# Autodesk Inventor assembly: Wheel Assembly
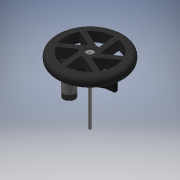
[picture p0: Inventor's stored thumbnail of the model, 180x180]
Saved by Autodesk Inventor 2017 (Build 210142000, 142)
## iProperties
Created: 2018-10-18
Part Number: Wheel Assembly
Document SubType Name: Assembly
Designer: Dell
Author: Dell
## Documents named in this file (8)
- C:\Users\Dell\Documents\GitHub\tr2\Wheel Assembly\Wheel Assembly.iam
- C:\Users\Dell\Documents\GitHub\tr2\Wheel Assembly\8mm Shaft.ipt
- C:\Users\Dell\Documents\GitHub\tr2\Wheel Assembly\Scooter Wheel.ipt
- C:\Users\Dell\Documents\GitHub\tr2\Wheel Assembly\WA01.ipt
- C:\Users\Dell\Documents\GitHub\tr2\Wheel Assembly\Wheel Assembly\Design Accelerator\Spur Gears1.iam
- C:\Users\Dell\Documents\GitHub\tr2\Base\37d-gearmotor-50-70-encoder.ipt
- C:\Users\Dell\Documents\GitHub\tr2\Wheel Assembly\22x8x8mm Bearing.ipt
- C:\Users\Dell\Documents\GitHub\tr2\Wheel Assembly\6mm Mounting Hub, thin.ipt
## Components (11 placed, 7 different names)
1. Scooter Wheel:1 — Mate:8, Flush:1, Mate:25, Mate:26, Mate:27, Mate:28
2. WA01:1 — Mate:2, Mate:9, Mate:10, Mate:11, Mate:24, Mate:31, Mate:33
3. 8mm Shaft:2 — Mate:2, Flush:1, Mate:16, Mate:18, Mate:23, Mate:29, Mate:30
4. Spur Gears:1 [sub-assembly] — Mate:8, Mate:17, Mate:19, Mate:21, Mate:22, Mate:30, Mate:31, Mate:32, Mate:33
5. 37d-gearmotor-50-70-encoder:1 — Mate:9, Mate:10, Mate:11, Mate:20, Mate:32
6. 22x8x8mm Bearing:1 — Mate:16, Mate:17
7. 22x8x8mm Bearing:2 — Mate:18, Mate:19
8. 6mm Mounting Hub, thin:1 — Mate:20, Mate:21, Mate:22
9. 22x8x8mm Bearing:3 — Mate:23, Mate:24
10. 22x8x8mm Bearing:4 — Mate:25, Mate:26
11. 22x8x8mm Bearing:5 — Mate:27, Mate:28, Mate:29
## Relationships (24: Mate 23, Flush 1)
- Mate:2: WA01:1 ↔ 8mm Shaft:2
- Mate:8: Scooter Wheel:1 ↔ Spur Gears:1
- Flush:1: Scooter Wheel:1 ↔ 8mm Shaft:2
- Mate:9: WA01:1 ↔ 37d-gearmotor-50-70-encoder:1
- Mate:10: WA01:1 ↔ 37d-gearmotor-50-70-encoder:1
- Mate:11: WA01:1 ↔ 37d-gearmotor-50-70-encoder:1
- Mate:16: 8mm Shaft:2 ↔ 22x8x8mm Bearing:1
- Mate:17: Spur Gears:1 ↔ 22x8x8mm Bearing:1
- Mate:18: 8mm Shaft:2 ↔ 22x8x8mm Bearing:2
- Mate:19: Spur Gears:1 ↔ 22x8x8mm Bearing:2
- Mate:20: 37d-gearmotor-50-70-encoder:1 ↔ 6mm Mounting Hub, thin:1
- Mate:21: Spur Gears:1 ↔ 6mm Mounting Hub, thin:1
- Mate:22: Spur Gears:1 ↔ 6mm Mounting Hub, thin:1
- Mate:23: 8mm Shaft:2 ↔ 22x8x8mm Bearing:3
- Mate:24: WA01:1 ↔ 22x8x8mm Bearing:3
- Mate:25: Scooter Wheel:1 ↔ 22x8x8mm Bearing:4
- Mate:26: Scooter Wheel:1 ↔ 22x8x8mm Bearing:4
- Mate:27: Scooter Wheel:1 ↔ 22x8x8mm Bearing:5
- Mate:28: Scooter Wheel:1 ↔ 22x8x8mm Bearing:5
- Mate:29: 8mm Shaft:2 ↔ 22x8x8mm Bearing:5
- Mate:30: 8mm Shaft:2 ↔ Spur Gears:1
- Mate:31: WA01:1 ↔ Spur Gears:1
- Mate:32: Spur Gears:1 ↔ 37d-gearmotor-50-70-encoder:1
- Mate:33: WA01:1 ↔ Spur Gears:1
